# Autodesk Inventor assembly: BASE
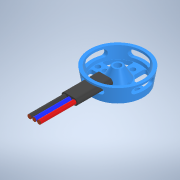
[picture p0: Inventor's stored thumbnail of the model, 180x180]
Saved by Autodesk Inventor 2022 (Build 260153000, 153)
## iProperties
Created: 2022-07-28
Part Number: BASE
Document SubType Name: Assembly
Designer: Nathan Cai
Author: Nathan Cai
## Documents named in this file (3)
- C:\Users\Nathan Cai\Documents\Inventor\Asorted Parts\Hobbyhh D3530 910KV\BASE.iam
- C:\Users\Nathan Cai\Documents\Inventor\Asorted Parts\Hobbyhh D3530 910KV\BODY.ipt
- C:\Users\Nathan Cai\Documents\Inventor\Asorted Parts\Hobbyhh D3530 910KV\SLEEVE.ipt
## Components (2 placed, 2 different names)
1. BODY:1 — Mate:1, Mate:2, Tangent:1
2. SLEEVE:1 — Mate:1, Mate:2, Tangent:1
## Relationships (3: Mate 2, Tangent 1)
- Mate:1: BODY:1 ↔ SLEEVE:1
- Mate:2 (-2 mm): BODY:1 ↔ SLEEVE:1
- Tangent:1: BODY:1 ↔ SLEEVE:1
